# Autodesk Inventor assembly: 094-DPK
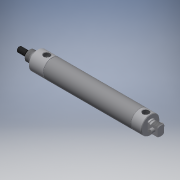
[picture p0: Inventor's stored thumbnail of the model, 180x180]
Saved by Autodesk Inventor 2019.4 (Build 234330000, 330)
## iProperties
Category: PARTsolutions
Company: BIMBA
Created: 2020-02-04
Part Number: 094-DPK
Catalog Web Link: www.cadenas.de
Description: Original Line Standard Air Cylinders-Standard Air Cylinders
Vendor: BIMBA
Document SubType Name: Assembly
Designer: psadmin
Manufacturer: BIMBA
Mass: 57.7574 g
Surface Area: 420.382 cm^2
Volume: 57.7574 cm^3
Density: 1 g/cm^3
PSOL_IDENT_0: {$CADENAS_DATA\23d-libs\bimba\bimba_brand\bimba_imperial\bimba_full_line\original_line_cylinders\sta
PSOL_IDENT_1: ndard_air_cylinders\standard_air_cylinder_asmtab.prj},322 {VTYP=3D},{STYP=ASSTAB},{NB=094-DPK},{LINA=
PSOL_IDENT_2: 094-DPK},{NN=Original Line Standard Air Cylinders},{DATE=22.01.2020 09:07:35},{GEOMDATE=24.10.2019 0
PSOL_IDENT_3: 9:09:47},{VERSION=},{LINEID=10},{WBVAR=STROKE,ACTING,MNT,DER,NR,BM,CO,OO,VO,M,EE,EEL,K,Q,Y,G,T,HL,B,
PSOL_IDENT_4: H,SER,SR,NT,W,STPT1,STPT2,STPT3,STPT4,MB,PB,PRC,TB,MN},{WBNUMERIC=STROKE,EEL}  {NB=094-DPK},{LINA=09
PSOL_IDENT_5: 4-DPK},{KT=DUMMY},{PN=094-DPK},{PNC=094-DPK},{PNA=(NO ACCESSORIES)},{DASH=-},{BORE1=1.06250000},{BOR
PSOL_IDENT_6: E=1 1/16\" (09)},{BOREPN=09},{STROKE=4.000},{STROKEALG=[0.011:50/0.001]},{STROKE1=4.000},{ACTING=D},
PSOL_IDENT_7: {ACTINGALG= '' , 'Single Acting' , 'R' , 'Reverse Single Acting (R)' , 'D' , 'Double Acting (D)' },{
PSOL_IDENT_8: ACTINGPN=D},{MNT=P},{MNTALG= '' , 'Front Nose Mounting' , 'P' , 'Rear Pivot Mounting (P)' , 'X' , 'U
PSOL_IDENT_9: niversal Pivot Mounting or Double End Mounting (X)' , 'BF' , 'Front Block Mounting (BF)' , 'BR' , 'R
PSOL_IDENT_10: ear Block Mounting for Vertical Positioning (BR)' , 'BFT' , 'Front Block Trunnion Mounting (BFT)' , '
PSOL_IDENT_11: BRT' , 'Rear Block Trunnion Mounting (BRT)' },{TYPE=},{MNTPN=P},{DER=},{DERALG= '' , 'N/A' },{NR=},{
PSOL_IDENT_12: NRALG= '' , 'N/A' },{NRPN=},{BM=},{BMALG= '' , 'N/A' },{BMPN=},{CO=},{COALG= '' , 'N/A' },{OO=},{OOA
PSOL_IDENT_13: LG= '', 'N/A' },{OOPN=},{VO=Z},{VOALG= 'Z' , 'N/A' },{VOPN=},{OOVOPN=},{M=},{MALG= '', 'Without Magn
PSOL_IDENT_14: et', 'M', 'With Magnet' },{EE=},{EEL=0.000},{EEMAX=46.0000},{EEALG= '', 'Without Extra Extension', '
PSOL_IDENT_15: EE', 'With Extra Extension' },{EELALG=0},{EEPN=},{EEPN1=0.000},{K=K},{KALG= '', 'Standard' , 'K' , '
PSOL_IDENT_16: Ports Rotated 90deg K' },{KPN=K},{Q=},{QALG= '' , 'N/A' },{QPN=},{Y=},{YALG= '' , 'Without Pivot Bus
PSOL_IDENT_17: hing' , 'Y' , 'With Pivot Bushing' },{YPN=},{YCON=},{F=},{FALG= '', 'Non-Coated (Standard)', 'F', 'M
PSOL_IDENT_18: olycoated' },{FPN=},{G=},{GPN=},{GPN99=},{T=},{TALG= '' , 'Standard -20° to 200°F (-29° to 95°C)' , '
PSOL_IDENT_19: N' , 'Low Temperature' , 'V' , 'High Temperature' },{NPN=},{VPN=},{HL=},{HLALG= '' , 'Without Low Pr
PSOL_IDENT_20: essure Hydraulic' , 'HL' , 'With Low Pressure Hydraulic' },{B=},{BALG= '', 'W/out Bumpers' , 'B' , '
PSOL_IDENT_21: W/ Bumpers' },{BPN=},{H=},{HALG= '', 'N/A' },{HPN=},{SER=},{SERALG= '' , 'Without Spring Extend/Retu
PSOL_IDENT_22: rn' , 'JS' , 'With Spring Return' , 'JR' , 'With Spring Extend' },{SR=C},{SRALG= 'C' , 'Standard Bla
PSOL_IDENT_23: ckened Carbon Steel' , 'SR' , 'Stainless Steel [SR]' },{SRPN=},{SRCON=1},{NT=},{NTPN=},{W=},{WALG= ''
PSOL_IDENT_24: , 'Without Wiper' , 'W' , 'With Wiper' },{WPN=},{E=},{EALG= '' , 'Standard Seals/Lube' , 'E' , 'Non
PSOL_IDENT_25: -Lube Seals/Lube' },{EPN=},{ST=},{STALG= '' , 'N/A' },{STPT1=},{STPT1ALG= '' , 'N/A' },{STPT2=},{STP
PSOL_IDENT_26: T2ALG= '' , 'N/A' },{STPT3=},{STPT3ALG= '' , 'N/A' },{STPT4=},{STPT4ALG= '' , 'N/A' },{STPN=},{MB=},
PSOL_IDENT_27: {MBALG= '' , 'N/A' },{MBPN=},{MBPNALL=},{MBPNALLREAR=},{PB=},{PBALG= '' , 'Without Pivot Bracket' , '
PSOL_IDENT_28: D-167' , 'D-167' },{PBPN=},{PBPNALL=D-167},{PRC=},{PRCALG= '' , 'W/out Pivot Rod Clevis' , 'F,D-166-
PSOL_IDENT_29: 1' , 'D-166-1 (front)' },{PRCPN=},{PRCPNALL=D-166-1},{TB=},{TBALG= '' , 'N/A' },{TBPN=},{TBPNALL=},{
PSOL_IDENT_30: MN=},{MNALG= '' , 'Without Mounting Nut' , 'F,D-9' , 'D-9 (front)' , 'R,D-9' , 'D-9 (rear)', '2x,D-9'
PSOL_IDENT_31: , 'D-9 (front & rear)' },{MNPN=},{MNCONF=},{MNCONR=},{TLEN=5.3185},{FRAC=22.8400},{RGCON=},{RGDACCO
PSOL_IDENT_32: N=R},{RHCON=P},{RHCON1=P},{RHCONON=1},{RHACCON=},{FNUTCON=0},{RNUTCON=0},{FNUTPN=D-9},{RNUTPN=D-9},{
PSOL_IDENT_33: FNUTTRANS=0.0000},{RNUTTRANS=0.0000},{VHOLECON=0},{A1=1.6250},{A1N=1.0000},{A1P=1.6250},{A1B=1.8750}
PSOL_IDENT_34: ,{A4=0.2525},{A4N=0.3750},{A4P=0.2525},{A5=0.0300},{A1H=1.5},{A1NH=0.6250},{A1PH=1.5000},{A1BH=1.125
PSOL_IDENT_35: 0},{A1SH=1.1250},{A2H=0.2500},{A2NH=0.2500},{LENGTH=3.8400},{LENGTH1=3.8400},{LENGTH2=4.1000},{MUL=4
PSOL_IDENT_36: .0000},{MUL11=4.0000},{MUL22=10.24},{MUL33=6.2400},{MUL2=4.0000},{MUL211=4.0000},{MUL222=2.5600},{MU
PSOL_IDENT_37: L233=1.5600},{SSS=8.0000},{RGLEN=1.4025},{RHLEN=0.9990},{SSS1=5.0000},{A13=1.2190},{DIF=0.1200},{G5=
PSOL_IDENT_38: 0.7180},{ON=0},{SSADD=0.0000},{BADD=0.0000},{MADD=0.0000},{NVADD=0.0000},{TRACKL=5.0285},{TRACKCON=D
PSOL_IDENT_39: -78527},{TRIMCON=0},{TRIMCON1=0},{PINCON=},{FSPACE=0.8134},{SPACE=0.1214},{TEXT=0.2125},{S1=1.2500},
PSOL_IDENT_40: {D1=1.1410},{D1N=1.1130},{D1B=1.1130},{D1P=1.1410},{FA=0.940},{RA=0.9400},{PPATH=standard_air_cylind
PSOL_IDENT_41: er_asmtpl.prj},{MATALGHTML=<b>Standard Original Line:</b><dl><dt>Rod:</dt><dd>- Stainless Steel</dd>
PSOL_IDENT_42: <dd>&nbsp;&nbsp;(5/16 9/16 Bores)</dd><dd>- High Strength Carbon Steel</dd><dd>&nbsp;&nbsp;(3/4 3 Bo
PSOL_IDENT_43: re)</dd><dd>- Stainless Steel</dd><dd>&nbsp;&nbsp;(X style DXP/DX/DXDE)</dd><dt>Bearings:</dt><dd>-
PSOL_IDENT_44: Sintered Bronze</dd><dt>Body:</dt><dd>- 304 Stainless Steel</dd><dt>End Caps:</dt><dd>- Aluminum</dd
PSOL_IDENT_45: ><dt>Seals:</dt><dd>- Buna N</dd></dl>},{ASSCFGPRA=09DP},{MBPNA=},{MNPNA=},{PRCPNA=},{ASSOPTACC=STPT
PSOL_IDENT_46: 4},{A=7.84},{HADD=0.0000},{WFL=0.125},{QADD=0.000},{QADD1=0.250},{TEST=4.0000},{MNTB=},{STDNUTF=0},{
PSOL_IDENT_47: STDNUTR=0},{STRK2D=0},{X2D=2},{STROKESW=4.000},{EESW=0.000},{FCD=0},{BCD=0},{RCD=0},{CUSTADD=3.000},
PSOL_IDENT_48: {FT=5/16-24 UNF-2A},{FT1=5/16-24 UNF-2A},{FT2=5/8-18 UNF-2A},{PORT=1/8 NPT},{FT11=5/8-18 UNF-2A},{FT
PSOL_IDENT_49: 12=5/8-18 UNF-2A},{B1=}
NN: Original Line Standard Air Cylinders
NT: Threaded (Standard)
NB: 094-DPK
NBSYN: $PNC.
LINA: 094-DPK
PN: 094-DPK
PNA: (NO ACCESSORIES)
BORE: 1 1/16" (09)
STROKE: 4
ACTING: Double Acting (D)
MNT: Rear Pivot Mounting (P)
DER: N/A
NR: N/A
BM: N/A
CO: N/A
OO: N/A
VO: N/A
M: Without Magnet
EE: Without Extra Extension
EEL: 0
K: Ports Rotated 90deg K
Q: N/A
Y: Without Pivot Bushing
G: Standard Lube
T: Standard -20° to 200°F (-29° to 95°C)
HL: Without Low Pressure Hydraulic
B: W/out Bumpers
H: N/A
SER: Without Spring Extend/Return
SR: Standard Blackened Carbon Steel
W: Without Wiper
STPT1: N/A
STPT2: N/A
STPT3: N/A
STPT4: N/A
MB: N/A
PB: Without Pivot Bracket
PRC: W/out Pivot Rod Clevis
TB: N/A
MN: Without Mounting Nut
A: 7.84
SUPPLIER: BIMBA
ARTICLENO: 094-DPK
BOMINFO: 094-DPK
CREATOR: CADENAS GmbH
Title: 094-DPK
Author: Cadenas PARTsolutions
Comments: Standard Air Cylinders
## Documents named in this file (7)
- T:\EIT\2020 Infinite Recharge\2020 ROBOT\COMMON PARTS\AIR CYLINDERS\094-DPK\AIS2018\094-DPK.iam
- T:\EIT\2020 Infinite Recharge\2020 ROBOT\COMMON PARTS\AIR CYLINDERS\094-DPK\AIS2018\094-DPCK0000000_0_dummy.ipt
- T:\EIT\2020 Infinite Recharge\2020 ROBOT\COMMON PARTS\AIR CYLINDERS\094-DPK\AIS2018\09RK000-0_rod_guide.ipt
- T:\EIT\2020 Infinite Recharge\2020 ROBOT\COMMON PARTS\AIR CYLINDERS\094-DPK\AIS2018\09R-5_31350C.ipt
- T:\EIT\2020 Infinite Recharge\2020 ROBOT\COMMON PARTS\AIR CYLINDERS\094-DPK\AIS2018\09P0K000_rear_head.ipt
- T:\EIT\2020 Infinite Recharge\2020 ROBOT\COMMON PARTS\AIR CYLINDERS\094-DPK\AIS2018\D-51.ipt
- T:\EIT\2020 Infinite Recharge\2020 ROBOT\COMMON PARTS\AIR CYLINDERS\094-DPK\AIS2018\C-094-DP0000_rod.ipt
## Components (6 placed, 6 different names)
1. 094-DPCK0000000_0_dummy:1
2. 09RK000-0_rod_guide:1 — Insert:1
3. 09R-5_31350C:1
4. 09P0K000_rear_head:1
5. D-51:1
6. C-094-DP0000_rod:1 — Insert:1
## Relationships (1: Insert 1)
- Insert:1: 09RK000-0_rod_guide:1 ↔ C-094-DP0000_rod:1
